# Autodesk Inventor assembly: Fan
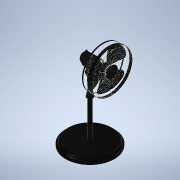
[picture p0: Inventor's stored thumbnail of the model, 180x180]
Saved by Autodesk Inventor 2022 (Build 260153000, 153)
## iProperties
Created: 2021-01-05
Part Number: Fan
Document SubType Name: Assembly
Designer: eahil
Author: eahil
## Documents named in this file (5)
- C:\Users\eng1-020\OneDrive - McMaster University\Winter term courses\Labs\Lab 8 Assignment (1)\Fan.iam
- C:\Users\eng1-020\OneDrive - McMaster University\Winter term courses\Labs\Lab 8 Assignment (1)\Base.ipt
- C:\Users\eng1-020\OneDrive - McMaster University\Winter term courses\Labs\Lab 8 Assignment (1)\Middle Section.ipt
- C:\Users\eng1-020\OneDrive - McMaster University\Winter term courses\Labs\Lab 8 Assignment (1)\Bracket.ipt
- C:\Users\eng1-020\OneDrive - McMaster University\Winter term courses\Labs\Lab 8 Assignment (1)\Fan Top.iam
## Components (4 placed, 4 different names)
1. Base:1 — Mate:1, Mate:2, Mate:3, Translation locked out
2. Middle Section:1 — Mate:1, Mate:2, Mate:3, Mate:4, Mate:5, Angle:2, Translation locked out
3. Bracket:1 — Mate:4, Mate:5, Mate:7, Mate:8, Angle:2, Angle:3, Horizontal bracket, Fan aligned
4. Fan Top:1 [sub-assembly] — Mate:7, Mate:8, Angle:3, Fan aligned
## Relationships (12: Mate 8, Angle 4)
- Mate:1: Base:1 ↔ Middle Section:1
- Mate:2: Base:1 ↔ Middle Section:1
- Mate:3: Base:1 ↔ Middle Section:1
- Mate:4: Middle Section:1 ↔ Bracket:1
- Mate:5: Middle Section:1 ↔ Bracket:1
- Mate:7: Bracket:1 ↔ Fan Top:1
- Mate:8: Bracket:1 ↔ Fan Top:1
- Angle:2 (0 deg): Middle Section:1 ↔ Bracket:1
- Translation locked out [Mate]: Base:1 ↔ Middle Section:1
- Angle:3 (-45 deg): Bracket:1 ↔ Fan Top:1
- Horizontal bracket [Angle] (0 deg): Bracket:1
- Fan aligned [Angle] (0 deg): Bracket:1 ↔ Fan Top:1
